# Autodesk Inventor assembly: holderWithGear
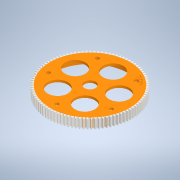
[picture p0: Inventor's stored thumbnail of the model, 180x180]
Saved by Autodesk Inventor 2022.1 (Build 261234000, 234)
## iProperties
Created: 2021-07-31
Part Number: holderWithGear
Document SubType Name: Assembly
Designer: robst
Author: robst
## Documents named in this file (3)
- C:\git\CAD-Development\robSteele\ShapeWays\TelescopeProjects\FilterWheel\holderWithGear.iam
- C:\git\CAD-Development\robSteele\ShapeWays\TelescopeProjects\FilterWheel\filterHolder.ipt
- C:\git\CAD-Development\robSteele\ShapeWays\TelescopeProjects\FilterWheel\filterWheelAssembly\Design Accelerator\Spur Gear13.ipt
## Components (2 placed, 2 different names)
1. filterHolder:1 — Insert:1
2. Spur Gear1:1 — Insert:1
## Relationships (1: Insert 1)
- Insert:1: filterHolder:1 ↔ Spur Gear1:1
